# Autodesk Inventor assembly: invacare assy
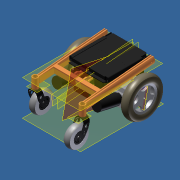
[picture p0: Inventor's stored thumbnail of the model, 180x180]
Saved by Autodesk Inventor 2012 (Build 160160000, 160)
## iProperties
Created: 2012-03-08
Part Number: invacare assy
Document SubType Name: Assembly
Designer: esv
Mass: 83979.9 g
Surface Area: 24308.3 cm^2
Volume: 48170.3 cm^3
Density: 1.7434 g/cm^3
Author: esv
## Documents named in this file (4)
- C:\Users\Edward\Documents\masters\CAD\Invacare\invacare assy.iam
- C:\Users\Edward\Documents\masters\CAD\Invacare\wheel.ipt
- C:\Users\Edward\Documents\masters\CAD\Invacare\frame_solid.iam
- C:\Users\Edward\Documents\masters\CAD\Invacare\caster assy.iam
## Components (5 placed, 3 different names)
1. frame_solid:1 [sub-assembly] — Insert:1, Insert:2, Insert:3, Insert:4
2. caster assy:1 [sub-assembly] — Insert:1
3. caster assy:2 [sub-assembly] — Insert:2
4. wheel:1 — Insert:3
5. wheel:2 — Insert:4
## Relationships (4: Insert 4)
- Insert:1: frame_solid:1 ↔ caster assy:1
- Insert:2: frame_solid:1 ↔ caster assy:2
- Insert:3: frame_solid:1 ↔ wheel:1
- Insert:4: frame_solid:1 ↔ wheel:2
